# Autodesk Inventor assembly: 2016-02-12-V17ShooterAndBase
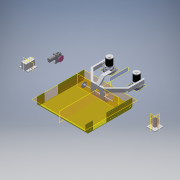
[picture p0: Inventor's stored thumbnail of the model, 180x180]
Saved by Autodesk Inventor 2016 SP1 (Build 200210100, 210)
## iProperties
Created: 2016-02-10
Part Number: 2016-02-12-V17ShooterAndBase
Document SubType Name: Assembly
Designer: steele
Author: steele
## Documents named in this file (6)
- C:\snobotics\CAD-Development\robSteele\SnoBotics2016\2016-02-08-RhinoTrackWithSheetBase\2016-02-12-V17ShooterAndBase.iam
- C:\snobotics\CAD-Development\robSteele\SnoBotics2016\RhinoBottomFloorOptions\SheetBottomFloorV01.ipt
- C:\snobotics\CAD-Development\robSteele\SnoBotics2016\2016-05-05-ShooterPrototype\SupportPlateMotorMountV01.ipt
- C:\snobotics\CAD-Development\robSteele\SnoBotics2016\2016-05-05-ShooterPrototype\SupportPlateWithPostOnlyV01.ipt
- C:\snobotics\CAD-Development\robSteele\SnoBotics2016\2016-05-05-ShooterPrototype\SnowBlowerMotorMountAndHub.iam
- C:\snobotics\CAD-Development\robSteele\SnoBotics2016\2016-05-05-ShooterPrototype\ShooterAssemblyForRobotV16.iam
## Components (5 placed, 5 different names)
1. SheetBottomFloorV01:1 — Mate:1, Flush:1
2. SupportPlateMotorMountV01:1
3. SupportPlateWithPostOnlyV01:1
4. SnowBlowerMotorMountAndHub:1 [sub-assembly]
5. ShooterAssemblyForRobotV16:1 [sub-assembly] — Mate:1, Mate:2
## Relationships (3: Mate 2, Flush 1)
- Mate:1: SheetBottomFloorV01:1 ↔ ShooterAssemblyForRobotV16:1
- Flush:1 (69.85 mm): SheetBottomFloorV01:1
- Mate:2: ShooterAssemblyForRobotV16:1
## Named parameters: distanceBaseToFloor = 50.8 mm
